# Autodesk Inventor assembly: parallel manipulator
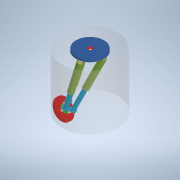
[picture p0: Inventor's stored thumbnail of the model, 180x180]
Saved by Autodesk Inventor 2020 (Build 240168000, 168)
## iProperties
Created: 2020-12-11
Part Number: parallel manipulator
Document SubType Name: Assembly
Designer: Vikki
Author: Vikki
## Documents named in this file (8)
- D:\borewell rescuebot\pll manipulator files\sps manipulator\parallel manipulator.iam
- D:\borewell rescuebot\pll manipulator files\sps manipulator\well.ipt
- D:\borewell rescuebot\pll manipulator files\sps manipulator\well maximum size.ipt
- D:\borewell rescuebot\pll manipulator files\sps manipulator\pll-base.ipt
- D:\borewell rescuebot\pll manipulator files\sps manipulator\pll-end eff.ipt
- D:\borewell rescuebot\pll manipulator files\sps manipulator\actuator assembly.iam
- D:\borewell rescuebot\pll manipulator files\sps manipulator\borewell max size.ipt
- D:\borewell rescuebot\pll manipulator files\sps manipulator\pin.ipt
## Components (9 placed, 7 different names)
1. well:1 — Flush:1, Mate:10
2. well maximum size:1 — Flush:1, Flush:2, Mate:2
3. pll-base:1 — Flush:2, Mate:2, Mate:3, Mate:4, Mate:5, Angle:1, Mate:9, Angle:2, Mate:12, Flush:3, Angle:3
4. pll-end eff:1 — Mate:6, Mate:7, Mate:8, Angle:1, Mate:9, Mate:10, Mate:11, Angle:2, Angle:3
5. actuator assembly:1 [sub-assembly] — Mate:3, Mate:7
6. actuator assembly:2 [sub-assembly] — Mate:4, Mate:6
7. actuator assembly:3 [sub-assembly] — Mate:5, Mate:8
8. pin:1 — Mate:11
9. borewell max size:1 — Mate:12, Flush:3
## Relationships (17: Mate 11, Flush 3, Angle 3)
- Flush:1: well:1 ↔ well maximum size:1
- Flush:2: well maximum size:1 ↔ pll-base:1
- Mate:2: well maximum size:1 ↔ pll-base:1
- Mate:3: pll-base:1 ↔ actuator assembly:1
- Mate:4: pll-base:1 ↔ actuator assembly:2
- Mate:5: pll-base:1 ↔ actuator assembly:3
- Mate:6: pll-end eff:1 ↔ actuator assembly:2
- Mate:7: pll-end eff:1 ↔ actuator assembly:1
- Mate:8: pll-end eff:1 ↔ actuator assembly:3
- Angle:1 (180 deg): pll-base:1 ↔ pll-end eff:1
- Mate:9: pll-base:1 ↔ pll-end eff:1
- Mate:10: well:1 ↔ pll-end eff:1
- Mate:11: pll-end eff:1 ↔ pin:1
- Angle:2 (0 deg): pll-base:1 ↔ pll-end eff:1
- Mate:12: pll-base:1 ↔ borewell max size:1
- Flush:3: pll-base:1 ↔ borewell max size:1
- Angle:3 (0 deg): pll-base:1 ↔ pll-end eff:1
